# Autodesk Inventor assembly: Lamp
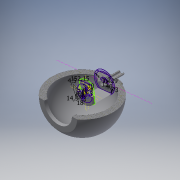
[picture p0: Inventor's stored thumbnail of the model, 180x180]
Saved by Autodesk Inventor 2018.2 (Build 222227000, 227)
## iProperties
Created: 2018-01-26
Part Number: Lamp
Material: Generisch
Document SubType Name: Assembly
Designer: JochenAlt
Author: JochenAlt
## Documents named in this file (4)
- D:\Projects\concretelamp\CAD\Lamp.iam
- D:\Projects\concretelamp\CAD\CableStrainRelief.ipt
- D:\Projects\concretelamp\CAD\Inlet.ipt
- D:\Projects\concretelamp\CAD\Lamp.ipt
## Components (3 placed, 3 different names)
1. Kabelzugentlastung:1 — Passend:1, Passend:2, Passend:3
2. V5 Inlet:1 — Passend:1, Passend:4
3. Lamp:1 — Passend:2, Passend:3, Passend:4
## Relationships (4: Mate 4)
- Passend:1 [Mate]: Kabelzugentlastung:1 ↔ V5 Inlet:1
- Passend:2 [Mate]: Kabelzugentlastung:1 ↔ Lamp:1
- Passend:3 [Mate] (0.5 mm): Kabelzugentlastung:1 ↔ Lamp:1
- Passend:4 [Mate] (0.5 mm): V5 Inlet:1 ↔ Lamp:1
